# Autodesk Inventor assembly: Assembly ebeam heater IS v0
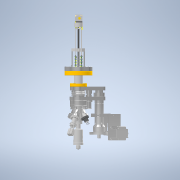
[picture p0: Inventor's stored thumbnail of the model, 180x180]
Saved by Autodesk Inventor 2020 (Build 240168000, 168)
## iProperties
Created: 2019-05-26
Part Number: Assembly ebeam heater IS v0
Document SubType Name: Assembly
Designer: isadmin
Mass: 1360.95 g
Surface Area: 5412.04 cm^2
Volume: 1345.69 cm^3
Density: 1.01134 g/cm^3
Author: isadmin
## Documents named in this file (32)
- C:\Users\ColinP\Documents\Inventor\ebeamheater v1\Assembly ebeam heater CP V1.iam
- Assembly ebeam heater IS v0.iam
- C:\Users\ColinP\Documents\Inventor\ebeamheater v1\block.ipt
- C:\Users\ColinP\Documents\Inventor\ebeamheater v1\Shutter.ipt
- C:\Users\ColinP\Documents\Inventor\ebeamheater v1\ceramic washer.ipt
- C:\Users\ColinP\Documents\Inventor\ebeamheater v1\Shielding.ipt
- C:\Users\ColinP\Documents\Inventor\ebeamheater v1\Bullet_v1_SiliconeSample.ipt
- C:\Users\ColinP\Documents\Inventor\ebeamheater v1\Bullet_v1_SiliconeSample_TopPart.ipt
- C:\Users\ColinP\Documents\Inventor\ebeamheater v1\670000.ipt
- C:\Users\ColinP\Documents\Inventor\ebeamheater v1\MCF275-FlgMplxr-Cr1A5_(53-321020-A).ipt
- C:\Users\ColinP\Documents\Inventor\ebeamheater v1\665501.ipt
- C:\Users\ColinP\Documents\Inventor\ebeamheater v1\rotatable rod table.ipt
- C:\Users\ColinP\Documents\Inventor\ebeamheater v1\updated table+legs.iam
- C:\Users\ColinP\Documents\Inventor\ebeamheater v1\square eyelet.ipt
- C:\Users\ColinP\Documents\Inventor\ebeamheater v1\buffer.ipt
- C:\Users\ColinP\Documents\Inventor\ebeamheater v1\4.5to2.75converotr.ipt
- C:\Users\ColinP\Documents\Inventor\ebeamheater v1\rotaryconnector.ipt
- C:\Users\ColinP\Documents\Inventor\ebeamheater v1\140007.ipt
- C:\Users\ColinP\Documents\Inventor\ebeamheater v1\bolt.ipt
- C:\Users\ColinP\Documents\Inventor\Content Center Files\R2020\en-US\ISO 4029\ISO 4029 - M2 x 2 - ISO.ipt
- C:\Users\ColinP\Documents\Inventor\ebeamheater v1\9312007.iam
- C:\Users\ColinP\Documents\Inventor\ebeamheater v1\eft0181032.ipt
- C:\Users\ColinP\Documents\Inventor\ebeamheater v1\filwasher.ipt
- C:\Users\ColinP\Documents\Inventor\ebeamheater v1\filament.ipt
- C:\Users\ColinP\Documents\Inventor\ebeamheater v1\fileholddub.ipt
- C:\Users\ColinP\Documents\Inventor\Content Center Files\R2020\en-US\ISO 4017(1)\ISO 4017 - M2.5 x 5 - ISO.ipt
- C:\Users\ColinP\Documents\Inventor\ebeamheater v1\flange 4_5 double_sided.ipt
- C:\Users\ColinP\Documents\Inventor\ebeamheater v1\450000.iam
- C:\Users\ColinP\Documents\Inventor\igor\stability copy2.ipt
- C:\Users\ColinP\Documents\Inventor\igor\stability copy.ipt
- C:\Users\ColinP\Documents\Inventor\Content Center Files\R2020\en-US\ISO 4032(2)\ISO 4032 - M3.5 - ISO.ipt
- C:\Users\ColinP\Documents\Inventor\Content Center Files\R2020\en-US\ISO 4032(2)\ISO 4032 - M3 - ISO.ipt
## Components (147 placed, 30 different names)
1. rotatable rod table:1 — Mate:48, Insert:171, Insert:173, Insert:174, Insert:175, Rigid:18, Insert:176, Insert:177, Insert:181, Mate:101, Mate:156, Insert:194, Insert:195
2. block for bullet:1
3. Shutter:1
4. ceramic washer:1
5. ceramic washer:2
6. ceramic washer:3
7. ceramic washer:4
8. Shielding:1
9. ceramic washer:5
10. ceramic washer:6
11. ceramic washer:7
12. ceramic washer:8
13. Bullet_v1_SiliconeSample:1
14. Bullet_v1_SiliconeSample_TopPart:1
15. rotation_670000:1 — Rotational:3, Rigid:18
16. MCF275-FlgMplxr-Cr1A5_(53-321020-A):1 — Rotational:3, Rigid:5, Rotational:5, Rotational:6, Rotational:10, Rigid:19
17. zstage_665501:1 — Rigid:8, Insert:137, Insert:138, Insert:139, Insert:140, Insert:141, Insert:142, Cylindrical:1
18. 140007:1 — Rigid:5, Rigid:8, Insert:131, Insert:132, Insert:133, Insert:134, Insert:135, Insert:136
19. updated table+legs:1 [sub-assembly] — Mate:48, Mate:72, Rigid:14, Insert:166, Rigid:16, Angle:1, Mate:106, Mate:142, Mate:143, Mate:144, Mate:145, Mate:146, Mate:147, Mate:162, Mate:163, Mate:164, Mate:166, Mate:168, Mate:170, Mate:172, Mate:174, Mate:176, Mate:178, Mate:180, Mate:182, Mate:184, Mate:186, Mate:188
20. buffer:4 — Insert:173
21. square eyelet:24 — Insert:210, Insert:214
22. square eyelet:25 — Mate:146, Insert:212, Insert:213
23. square eyelet:26 — Insert:211, Mate:185
24. buffer:5 — Insert:171
25. square eyelet:27 — Mate:142, Insert:206
26. square eyelet:28 — Insert:203, Insert:204
27. square eyelet:29 — Insert:202, Insert:205
28. buffer:6 — Insert:161, Insert:162, Insert:163, Insert:174
29. buffer:7 — Insert:176
30. square eyelet:33 — Insert:231, Insert:236
31. square eyelet:34 — Mate:147, Insert:233, Insert:234
32. square eyelet:35 — Insert:232, Insert:235
33. buffer:9 — Insert:177
34. square eyelet:39 — Insert:207, Mate:183
35. square eyelet:40 — Mate:144, Mate:181, Insert:208
36. square eyelet:41 — Mate:179, Insert:209
37. rotaryconnector:2 — Insert:149, Insert:150, Insert:151, Insert:152
38. 4.5to2.75converotr:1 — Cylindrical:1, Mate:99, Mate:100
39. square eyelet:49 — Insert:134
40. square eyelet:50 — Insert:135
41. square eyelet:51 — Insert:133
42. square eyelet:52 — Insert:131, Mate:72
43. square eyelet:53 — Insert:132
44. square eyelet:54 — Insert:136
45. bolt:1 — Insert:142
46. bolt:2 — Insert:138
47. bolt:3 — Insert:140
48. bolt:4 — Insert:139
49. bolt:5 — Insert:141
50. bolt:6 — Insert:137
51. buffer:10 — Insert:175
52. square eyelet:55 — Mate:143, Insert:197, Mate:177
53. square eyelet:56 — Insert:199, Insert:200
54. square eyelet:57 — Insert:198, Mate:175
55. 9312007:1 [sub-assembly] — Rotational:5
56. eft0181032:1 — Rotational:6
57. square eyelet:64 — Insert:162, Insert:227, Mate:189
58. square eyelet:65 — Insert:163, Insert:228, Mate:187
59. square eyelet:66 — Insert:161, Mate:145, Insert:229, Insert:230
60. filament:1 — Mate:126, Mate:127
61. filwasher:2 — Rigid:14, Insert:168, Mate:148
62. fileholddub:1 — Insert:166, Rigid:17, Rotational:9, Angle:1
63. filwasher:5 — Rotational:9, Insert:169, Mate:149
64. filwasher:6 — Rigid:17, Insert:170, Mate:127
65. filwasher:7 — Rigid:16, Insert:167, Mate:126
66. buffer:11 — Insert:178, Insert:179, Insert:180, Insert:181
67. square eyelet:67 — Insert:178, Mate:106, Mate:169, Mate:171
68. square eyelet:68 — Insert:179, Mate:167, Mate:173
69. square eyelet:69 — Insert:180, Mate:165, Insert:196
70. flange 4_5 double_sided:1 — Mate:99, Mate:100, Mate:101, Mate:161, Flush:3
71. ISO 4029 M2 x 2:1 — Insert:152
72. ISO 4029 M2 x 2:2 — Insert:150
73. ISO 4029 M2 x 2:3 — Insert:151
74. ISO 4029 M2 x 2:4 — Insert:149
75. ISO 4017 M2.5 x 5:1 — Insert:167
76. ISO 4017 M2.5 x 5:2 — Insert:168
77. ISO 4017 M2.5 x 5:3 — Insert:169
78. ISO 4017 M2.5 x 5:4 — Insert:170
79. filament:2 — Mate:148, Mate:149
80. 450000:1 [sub-assembly] — Rigid:19
81. 450000:2 [sub-assembly] — Rotational:10
82. stability copy2:1 — Mate:159, Insert:187, Mate:161, Flush:3
83. stability copy2:2 — Insert:185, Mate:160
84. stability copy2:3 — Mate:158, Insert:186
85. stability copy:1 — Mate:156, Mate:158, Insert:185, Insert:186, Mate:159, Insert:187, Mate:160
86. buffer:12 — Insert:194
87. square eyelet:70 — Insert:215, Insert:220
88. square eyelet:71 — Mate:162, Insert:216, Insert:219
89. square eyelet:72 — Insert:217, Insert:218
90. buffer:13 — Insert:195
91. square eyelet:73 — Insert:221, Insert:226
92. square eyelet:74 — Mate:163, Insert:222, Insert:225
93. square eyelet:75 — Insert:223, Insert:224
94. ISO 4032 M3.5:1 — Mate:164, Mate:165
95. ISO 4032 M3.5:2 — Mate:166, Mate:167
96. ISO 4032 M3.5:3 — Mate:168, Mate:169
97. ISO 4032 M3.5:4 — Mate:170, Mate:171
98. ISO 4032 M3.5:5 — Mate:172, Mate:173
99. ISO 4032 M3:1 — Insert:196
100. ISO 4032 M3:2 — Insert:197
101. ISO 4032 M3:3 — Insert:198
102. ISO 4032 M3:4 — Insert:199
103. ISO 4032 M3:5 — Insert:200
104. ISO 4032 M3.5:6 — Mate:174, Mate:175
105. ISO 4032 M3.5:7 — Mate:176, Mate:177, Insert:201
106. ISO 4032 M3.5:8 — Insert:201
107. ISO 4032 M3:6 — Insert:202
108. ISO 4032 M3:7 — Insert:203
109. ISO 4032 M3:8 — Insert:204
110. ISO 4032 M3:9 — Insert:205
111. ISO 4032 M3:10 — Insert:206
112. ISO 4032 M3:11 — Insert:207
113. ISO 4032 M3.5:9 — Mate:178, Mate:179
114. ISO 4032 M3.5:10 — Mate:180, Mate:181
115. ISO 4032 M3:12 — Insert:208
116. ISO 4032 M3:13 — Insert:209
117. ISO 4032 M3.5:11 — Mate:182, Mate:183
118. ISO 4032 M3:14 — Insert:210
119. ISO 4032 M3:15 — Insert:211
120. ISO 4032 M3:16 — Insert:212
121. ISO 4032 M3:17 — Insert:213
122. ISO 4032 M3.5:12 — Mate:184, Mate:185
123. ISO 4032 M3:18 — Insert:214
124. ISO 4032 M3:19 — Insert:215
125. ISO 4032 M3:20 — Insert:216
126. ISO 4032 M3:21 — Insert:217
127. ISO 4032 M3:22 — Insert:218
128. ISO 4032 M3:23 — Insert:219
129. ISO 4032 M3:24 — Insert:220
130. ISO 4032 M3:25 — Insert:221
131. ISO 4032 M3:26 — Insert:222
132. ISO 4032 M3:27 — Insert:223
133. ISO 4032 M3:28 — Insert:224
134. ISO 4032 M3:29 — Insert:225
135. ISO 4032 M3:30 — Insert:226
136. ISO 4032 M3:31 — Insert:227
137. ISO 4032 M3:32 — Insert:228
138. ISO 4032 M3:33 — Insert:229
139. ISO 4032 M3:34 — Insert:230
140. ISO 4032 M3.5:13 — Mate:186, Mate:187
141. ISO 4032 M3.5:14 — Mate:188, Mate:189
142. ISO 4032 M3:35 — Insert:231
143. ISO 4032 M3:36 — Insert:232
144. ISO 4032 M3:37 — Insert:233
145. ISO 4032 M3:38 — Insert:234
146. ISO 4032 M3:39 — Insert:235
147. ISO 4032 M3:40 — Insert:236
## Relationships (192: Insert 104, Mate 71, WeldJoint 7, RevoluteJoint 5, Flush 3, Angle 1, CylindricalJoint 1)
- [Mate]: block for bullet:1 ↔ Shutter:1
- [Mate]: block for bullet:1 ↔ Shutter:1
- [Mate]: block for bullet:1 ↔ Shutter:1
- [Mate]: block for bullet:1 ↔ ceramic washer:2
- [Mate]: block for bullet:1 ↔ ceramic washer:2
- [Mate]: block for bullet:1 ↔ ceramic washer:1
- [Mate]: block for bullet:1 ↔ ceramic washer:1
- [Mate]: block for bullet:1 ↔ ceramic washer:4
- [Mate]: block for bullet:1 ↔ ceramic washer:4
- [Mate]: block for bullet:1 ↔ ceramic washer:3
- [Mate]: block for bullet:1 ↔ ceramic washer:3
- [Mate]: ceramic washer:1 ↔ Shielding:1
- [Flush]: block for bullet:1 ↔ Shielding:1
- [Flush]: block for bullet:1 ↔ Shielding:1
- [Mate]: block for bullet:1 ↔ ceramic washer:5
- [Mate]: block for bullet:1 ↔ ceramic washer:5
- [Mate]: block for bullet:1 ↔ ceramic washer:6
- [Mate]: block for bullet:1 ↔ ceramic washer:6
- [Mate]: block for bullet:1 ↔ ceramic washer:7
- [Mate]: block for bullet:1 ↔ ceramic washer:7
- [Mate]: block for bullet:1 ↔ ceramic washer:8
- [Mate]: block for bullet:1 ↔ ceramic washer:8
- [Mate] (0.0254 mm): Bullet_v1_SiliconeSample:1 ↔ Bullet_v1_SiliconeSample_TopPart:1
- [Mate]: Bullet_v1_SiliconeSample:1 ↔ Bullet_v1_SiliconeSample_TopPart:1
- [Insert]: block for bullet:1 ↔ Bullet_v1_SiliconeSample:1
- [Insert]: rotatable rod table:1 ↔ block for bullet:1
- [Insert]: rotatable rod table:1 ↔ block for bullet:1
- [Insert]: buffer:4 ↔ square eyelet:25
- [Insert]: buffer:4 ↔ square eyelet:24
- [Insert]: buffer:4 ↔ square eyelet:26
- [Insert]: buffer:5 ↔ square eyelet:28
- [Insert]: buffer:5 ↔ square eyelet:27
- [Insert]: buffer:5 ↔ square eyelet:29
- [Insert]: buffer:7 ↔ square eyelet:34
- [Insert]: buffer:7 ↔ square eyelet:33
- [Insert]: buffer:7 ↔ square eyelet:35
- [Insert]: buffer:9 ↔ square eyelet:40
- [Insert]: buffer:9 ↔ square eyelet:39
- [Insert]: buffer:9 ↔ square eyelet:41
- Mate:48: rotatable rod table:1 ↔ updated table+legs:1
- Rotational:3 [RevoluteJoint]: rotation_670000:1 ↔ MCF275-FlgMplxr-Cr1A5_(53-321020-A):1
- Rigid:5 [WeldJoint]: MCF275-FlgMplxr-Cr1A5_(53-321020-A):1 ↔ 140007:1
- Rigid:8 [WeldJoint]: zstage_665501:1 ↔ 140007:1
- Insert:131: 140007:1 ↔ square eyelet:52
- Insert:132: 140007:1 ↔ square eyelet:53
- Insert:133: 140007:1 ↔ square eyelet:51
- Insert:134: 140007:1 ↔ square eyelet:49
- Insert:135: 140007:1 ↔ square eyelet:50
- Insert:136: 140007:1 ↔ square eyelet:54
- Insert:137: zstage_665501:1 ↔ bolt:6
- Insert:138: zstage_665501:1 ↔ bolt:2
- Insert:139: zstage_665501:1 ↔ bolt:4
- Insert:140: zstage_665501:1 ↔ bolt:3
- Insert:141: zstage_665501:1 ↔ bolt:5
- Insert:142: zstage_665501:1 ↔ bolt:1
- [Insert]: buffer:10 ↔ square eyelet:56
- [Insert]: buffer:10 ↔ square eyelet:55
- [Insert]: buffer:10 ↔ square eyelet:57
- Insert:149: rotaryconnector:2 ↔ ISO 4029 M2 x 2:4
- Insert:150: rotaryconnector:2 ↔ ISO 4029 M2 x 2:2
- Insert:151: rotaryconnector:2 ↔ ISO 4029 M2 x 2:3
- Insert:152: rotaryconnector:2 ↔ ISO 4029 M2 x 2:1
- Rotational:5 [RevoluteJoint]: MCF275-FlgMplxr-Cr1A5_(53-321020-A):1 ↔ 9312007:1
- Rotational:6 [RevoluteJoint]: MCF275-FlgMplxr-Cr1A5_(53-321020-A):1 ↔ eft0181032:1
- Mate:72: updated table+legs:1 ↔ square eyelet:52
- Insert:161: buffer:6 ↔ square eyelet:66
- Insert:162: buffer:6 ↔ square eyelet:64
- Insert:163: buffer:6 ↔ square eyelet:65
- Rigid:14 [WeldJoint]: updated table+legs:1 ↔ filwasher:2
- Insert:166 (-7.62 mm): updated table+legs:1 ↔ fileholddub:1
- Rigid:16 [WeldJoint]: updated table+legs:1 ↔ filwasher:7
- Rigid:17 [WeldJoint]: fileholddub:1 ↔ filwasher:6
- Rotational:9 [RevoluteJoint]: fileholddub:1 ↔ filwasher:5
- Insert:167: filwasher:7 ↔ ISO 4017 M2.5 x 5:1
- Insert:168: filwasher:2 ↔ ISO 4017 M2.5 x 5:2
- Insert:169: filwasher:5 ↔ ISO 4017 M2.5 x 5:3
- Insert:170: filwasher:6 ↔ ISO 4017 M2.5 x 5:4
- Insert:171 (163.83 mm): rotatable rod table:1 ↔ buffer:5
- Insert:173 (187.96 mm): rotatable rod table:1 ↔ buffer:4
- Insert:174 (223.52 mm): rotatable rod table:1 ↔ buffer:6
- Insert:175 (152.4 mm): rotatable rod table:1 ↔ buffer:10
- Angle:1 (180 deg): updated table+legs:1 ↔ fileholddub:1
- Rigid:18 [WeldJoint]: rotatable rod table:1 ↔ rotation_670000:1
- Insert:176 (234.95 mm): rotatable rod table:1 ↔ buffer:7
- Insert:177 (175.26 mm): rotatable rod table:1 ↔ buffer:9
- Insert:178: buffer:11 ↔ square eyelet:67
- Insert:179: buffer:11 ↔ square eyelet:68
- Insert:180: buffer:11 ↔ square eyelet:69
- Insert:181 (140.97 mm): rotatable rod table:1 ↔ buffer:11
- Cylindrical:1: zstage_665501:1 ↔ 4.5to2.75converotr:1
- Mate:99: 4.5to2.75converotr:1 ↔ flange 4_5 double_sided:1
- Mate:100: 4.5to2.75converotr:1 ↔ flange 4_5 double_sided:1
- Mate:101: rotatable rod table:1 ↔ flange 4_5 double_sided:1
- Mate:106: updated table+legs:1 ↔ square eyelet:67
- Mate:126: filament:1 ↔ filwasher:7
- Mate:127: filament:1 ↔ filwasher:6
- Mate:142: updated table+legs:1 ↔ square eyelet:27
- Mate:143: updated table+legs:1 ↔ square eyelet:55
- Mate:144: updated table+legs:1 ↔ square eyelet:40
- Mate:145: updated table+legs:1 ↔ square eyelet:66
- Mate:146: updated table+legs:1 ↔ square eyelet:25
- Mate:147: updated table+legs:1 ↔ square eyelet:34
- Mate:148: filwasher:2 ↔ filament:2
- Mate:149: filwasher:5 ↔ filament:2
- Rotational:10 [RevoluteJoint]: MCF275-FlgMplxr-Cr1A5_(53-321020-A):1 ↔ 450000:2
- Rigid:19 [WeldJoint]: MCF275-FlgMplxr-Cr1A5_(53-321020-A):1 ↔ 450000:1
- Mate:156: rotatable rod table:1 ↔ stability copy:1
- Mate:158: stability copy2:3 ↔ stability copy:1
- Insert:185: stability copy2:2 ↔ stability copy:1
- Insert:186: stability copy2:3 ↔ stability copy:1
- Mate:159: stability copy2:1 ↔ stability copy:1
- Insert:187: stability copy2:1 ↔ stability copy:1
- Mate:160: stability copy2:2 ↔ stability copy:1
- Mate:161: flange 4_5 double_sided:1 ↔ stability copy2:1
- Flush:3: flange 4_5 double_sided:1 ↔ stability copy2:1
- [Insert]: buffer:12 ↔ square eyelet:72
- [Insert]: buffer:12 ↔ square eyelet:70
- [Insert]: buffer:12 ↔ square eyelet:71
- [Insert]: buffer:13 ↔ square eyelet:75
- [Insert]: buffer:13 ↔ square eyelet:73
- [Insert]: buffer:13 ↔ square eyelet:74
- Mate:162: updated table+legs:1 ↔ square eyelet:71
- Mate:163: updated table+legs:1 ↔ square eyelet:74
- Insert:194 (-168.91 mm): rotatable rod table:1 ↔ buffer:12
- Insert:195 (-156.845 mm): rotatable rod table:1 ↔ buffer:13
- Mate:164: updated table+legs:1 ↔ ISO 4032 M3.5:1
- Mate:165: square eyelet:69 ↔ ISO 4032 M3.5:1
- Mate:166: updated table+legs:1 ↔ ISO 4032 M3.5:2
- Mate:167: square eyelet:68 ↔ ISO 4032 M3.5:2
- Mate:168: updated table+legs:1 ↔ ISO 4032 M3.5:3
- Mate:169: square eyelet:67 ↔ ISO 4032 M3.5:3
- Mate:170: updated table+legs:1 ↔ ISO 4032 M3.5:4
- Mate:171: square eyelet:67 ↔ ISO 4032 M3.5:4
- Mate:172: updated table+legs:1 ↔ ISO 4032 M3.5:5
- Mate:173: square eyelet:68 ↔ ISO 4032 M3.5:5
- Insert:196: square eyelet:69 ↔ ISO 4032 M3:1
- Insert:197: square eyelet:55 ↔ ISO 4032 M3:2
- Insert:198: square eyelet:57 ↔ ISO 4032 M3:3
- Insert:199: square eyelet:56 ↔ ISO 4032 M3:4
- Insert:200: square eyelet:56 ↔ ISO 4032 M3:5
- Mate:174: updated table+legs:1 ↔ ISO 4032 M3.5:6
- Mate:175: square eyelet:57 ↔ ISO 4032 M3.5:6
- Mate:176: updated table+legs:1 ↔ ISO 4032 M3.5:7
- Mate:177: square eyelet:55 ↔ ISO 4032 M3.5:7
- Insert:201: ISO 4032 M3.5:7 ↔ ISO 4032 M3.5:8
- Insert:202: square eyelet:29 ↔ ISO 4032 M3:6
- Insert:203: square eyelet:28 ↔ ISO 4032 M3:7
- Insert:204: square eyelet:28 ↔ ISO 4032 M3:8
- Insert:205: square eyelet:29 ↔ ISO 4032 M3:9
- Insert:206: square eyelet:27 ↔ ISO 4032 M3:10
- Insert:207: square eyelet:39 ↔ ISO 4032 M3:11
- Mate:178: updated table+legs:1 ↔ ISO 4032 M3.5:9
- Mate:179: square eyelet:41 ↔ ISO 4032 M3.5:9
- Mate:180: updated table+legs:1 ↔ ISO 4032 M3.5:10
- Mate:181: square eyelet:40 ↔ ISO 4032 M3.5:10
- Insert:208: square eyelet:40 ↔ ISO 4032 M3:12
- Insert:209: square eyelet:41 ↔ ISO 4032 M3:13
- Mate:182: updated table+legs:1 ↔ ISO 4032 M3.5:11
- Mate:183: square eyelet:39 ↔ ISO 4032 M3.5:11
- Insert:210: square eyelet:24 ↔ ISO 4032 M3:14
- Insert:211: square eyelet:26 ↔ ISO 4032 M3:15
- Insert:212: square eyelet:25 ↔ ISO 4032 M3:16
- Insert:213: square eyelet:25 ↔ ISO 4032 M3:17
- Mate:184: updated table+legs:1 ↔ ISO 4032 M3.5:12
- Mate:185: square eyelet:26 ↔ ISO 4032 M3.5:12
- Insert:214: square eyelet:24 ↔ ISO 4032 M3:18
- Insert:215: square eyelet:70 ↔ ISO 4032 M3:19
- Insert:216: square eyelet:71 ↔ ISO 4032 M3:20
- Insert:217: square eyelet:72 ↔ ISO 4032 M3:21
- Insert:218: square eyelet:72 ↔ ISO 4032 M3:22
- Insert:219: square eyelet:71 ↔ ISO 4032 M3:23
- Insert:220: square eyelet:70 ↔ ISO 4032 M3:24
- Insert:221: square eyelet:73 ↔ ISO 4032 M3:25
- Insert:222: square eyelet:74 ↔ ISO 4032 M3:26
- Insert:223: square eyelet:75 ↔ ISO 4032 M3:27
- Insert:224: square eyelet:75 ↔ ISO 4032 M3:28
- Insert:225: square eyelet:74 ↔ ISO 4032 M3:29
- Insert:226: square eyelet:73 ↔ ISO 4032 M3:30
- Insert:227: square eyelet:64 ↔ ISO 4032 M3:31
- Insert:228: square eyelet:65 ↔ ISO 4032 M3:32
- Insert:229: square eyelet:66 ↔ ISO 4032 M3:33
- Insert:230: square eyelet:66 ↔ ISO 4032 M3:34
- Mate:186: updated table+legs:1 ↔ ISO 4032 M3.5:13
- Mate:187: square eyelet:65 ↔ ISO 4032 M3.5:13
- Mate:188: updated table+legs:1 ↔ ISO 4032 M3.5:14
- Mate:189: square eyelet:64 ↔ ISO 4032 M3.5:14
- Insert:231: square eyelet:33 ↔ ISO 4032 M3:35
- Insert:232: square eyelet:35 ↔ ISO 4032 M3:36
- Insert:233: square eyelet:34 ↔ ISO 4032 M3:37
- Insert:234: square eyelet:34 ↔ ISO 4032 M3:38
- Insert:235: square eyelet:35 ↔ ISO 4032 M3:39
- Insert:236: square eyelet:33 ↔ ISO 4032 M3:40
## Named parameters: d75_d58 = 0 mm, d76_d19 = 0 mm, d77_d22_d25 = 0 mm, d78_d23_d26 = 0 mm, d79_d24_d35 = 0 mm, d80_d25_d36 = 0 mm, d81_d26_d37 = 0 mm, d82_d27_d38 = 0 mm, d83_d28_d39 = 0 mm, d84_d29_d40 = 0 mm, d85_d30_d41 = 0 mm, d86_d31_d42 = 0 mm, d87_d43 = 0 mm, d88_d44 = 0 mm, d89_d45 = 0 mm, d90_d46 = 0 mm, d91_d47 = 0 mm, d92_d48 = 0 mm, d93_d49 = 0 mm, d94_d50 = 0 mm, d95_d51 = 0 mm, d96_d52 = 0 mm, d97_d53 = 0 mm, d98_d56_d0 = 0.0254 mm, d99_d57_d1 = 0 mm, d148_d124_d114_d111 = 0 mm, d149_d125_d115_d112 = 0 mm, d150_d126_d116_d113 = 0 mm, d152_d124_d114_d111 = 0 mm, d153_d125_d115_d112 = 0 mm, d154_d126_d116_d113 = 0 mm, d163_d124_d114_d111 = 0 mm, d164_d125_d115_d112 = 0 mm, d165_d126_d116_d113 = 0 mm, d175_d111 = 0 mm, d176_d112 = 0 mm, d177_d113 = 0 mm, d314_d124_d114_d111 = 0 mm, d315_d125_d115_d112 = 0 mm, d316_d126_d116_d113 = 0 mm, d749_d445 = 0 mm, d750_d446 = 0 mm, d751_d447 = 0 mm, d752_d445 = 0 mm, d753_d446 = 0 mm, d754_d447 = 0 mm
